# Autodesk Inventor assembly: 00_Linear_rail_X
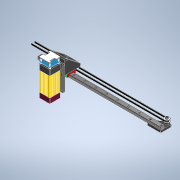
[picture p0: Inventor's stored thumbnail of the model, 180x180]
Saved by Autodesk Inventor 2022.2 (Build 262287010, 287A)
## iProperties
Created: 2022-05-03
Part Number: 00_Linear_rail_X
Document SubType Name: Assembly
Designer: MXBD
Author: MXBD
## Documents named in this file (13)
- D:\Laser_Engraver\CAD\Assembly\00_Linear_rail_X.iam
- D:\Laser_Engraver\CAD\Parts\02_mgn15h_Rail_450mm.ipt
- D:\Laser_Engraver\CAD\Parts\01_mgn15h_Bearing_Block.ipt
- D:\Laser_Engraver\CAD\Assembly\01_Laser_Assy.iam
- D:\Laser_Engraver\CAD\Parts\21_X_Pulley_holder.ipt
- D:\Laser_Engraver\CAD\Parts\23_Spacers_7.7mm.ipt
- D:\Laser_Engraver\CAD\Parts\10_GT2_Idler_Pulley_20_Teeth.ipt
- C:\Users\49152\Documents\Inventor\Content Center Files\R2022\de-DE\ISO 4762(2)\ISO 4762 - M5 x 30ISO.ipt
- C:\Users\49152\Documents\Inventor\Content Center Files\R2022\de-DE\ISO 4762(2)\ISO 4762 - M3 x 12ISO.ipt
- C:\Users\49152\Documents\Inventor\Content Center Files\R2022\de-DE\DIN 555\DIN 555-5 - M5.ipt
- C:\Users\49152\Documents\Inventor\Content Center Files\R2022\de-DE\ISO 4762(2)\ISO 4762 - M5 x 20ISO.ipt
- C:\Users\49152\Documents\Inventor\Content Center Files\R2022\de-DE\ISO 4762(2)\ISO 4762 - M3 x 8ISO.ipt
- D:\Laser_Engraver\CAD\Parts\20_Belt_490mm.ipt
## Components (18 placed, 12 different names)
1. 02_mgn15h_Rail_450mm:1 — Passend:1, Passend:2, Passend:6, Passend:7, Passend:8, Passend:15, Passend:16, Passend:17, Passend:18, Winkel:1, Passend:33, Fluchtend:1
2. 01_mgn15h_Bearing_Block:1 — Passend:1, Passend:2, Passend:3, Passend:4, Passend:5
3. 01_Laser_Assy:1 [sub-assembly] — Passend:3, Passend:4, Passend:5, Passend:21, Passend:22, Passend:23, Passend:24, Passend:25, Passend:26, Passend:27, Passend:28, Passend:29, Passend:30, Passend:31, Passend:32
4. 21_X_Pulley_holder:1 — Passend:6, Passend:7, Passend:8, Passend:9, Passend:10, Passend:20
5. 23_Spacers_7.7mm:1 — Passend:9, Passend:10, Passend:11, Passend:12
6. 10_GT2_Idler_Pulley_20_Teeth:1 — Passend:11, Passend:12, Passend:13, Passend:14, Passend:34
7. ISO 4762 M5 x 30:1 — Passend:13, Passend:14, Passend:19
8. ISO 4762 M3 x 12:1 — Passend:15, Passend:18
9. ISO 4762 M3 x 12:2 — Passend:16, Passend:17
10. DIN 555 - ersetzt durch DIN EN 24034 M5:1 — Passend:19, Passend:20
11. ISO 4762 M5 x 20:1 — Passend:21, Passend:23
12. ISO 4762 M5 x 20:2 — Passend:22, Passend:24
13. ISO 4762 M3 x 8:1 — Passend:25, Passend:31
14. ISO 4762 M3 x 8:2 — Passend:26, Passend:30
15. ISO 4762 M3 x 8:3 — Passend:27, Passend:32
16. ISO 4762 M3 x 8:4 — Passend:28, Passend:29
17. 20_Belt_490mm:2 — Passend:35, Fluchtend:2, Fluchtend:3
18. 20_Belt_490mm:3 — Winkel:1, Passend:33, Passend:34, Fluchtend:1, Passend:35, Fluchtend:2, Fluchtend:3
## Relationships (39: Mate 35, Flush 3, Angle 1)
- Passend:1 [Mate]: 02_mgn15h_Rail_450mm:1 ↔ 01_mgn15h_Bearing_Block:1
- Passend:2 [Mate]: 02_mgn15h_Rail_450mm:1 ↔ 01_mgn15h_Bearing_Block:1
- Passend:3 [Mate]: 01_mgn15h_Bearing_Block:1 ↔ 01_Laser_Assy:1
- Passend:4 [Mate]: 01_mgn15h_Bearing_Block:1 ↔ 01_Laser_Assy:1
- Passend:5 [Mate]: 01_mgn15h_Bearing_Block:1 ↔ 01_Laser_Assy:1
- Passend:6 [Mate]: 02_mgn15h_Rail_450mm:1 ↔ 21_X_Pulley_holder:1
- Passend:7 [Mate]: 02_mgn15h_Rail_450mm:1 ↔ 21_X_Pulley_holder:1
- Passend:8 [Mate]: 02_mgn15h_Rail_450mm:1 ↔ 21_X_Pulley_holder:1
- Passend:9 [Mate]: 21_X_Pulley_holder:1 ↔ 23_Spacers_7.7mm:1
- Passend:10 [Mate]: 21_X_Pulley_holder:1 ↔ 23_Spacers_7.7mm:1
- Passend:11 [Mate]: 23_Spacers_7.7mm:1 ↔ 10_GT2_Idler_Pulley_20_Teeth:1
- Passend:12 [Mate]: 23_Spacers_7.7mm:1 ↔ 10_GT2_Idler_Pulley_20_Teeth:1
- Passend:13 [Mate]: 10_GT2_Idler_Pulley_20_Teeth:1 ↔ ISO 4762 M5 x 30:1
- Passend:14 [Mate]: 10_GT2_Idler_Pulley_20_Teeth:1 ↔ ISO 4762 M5 x 30:1
- Passend:15 [Mate]: 02_mgn15h_Rail_450mm:1 ↔ ISO 4762 M3 x 12:1
- Passend:16 [Mate]: 02_mgn15h_Rail_450mm:1 ↔ ISO 4762 M3 x 12:2
- Passend:17 [Mate]: 02_mgn15h_Rail_450mm:1 ↔ ISO 4762 M3 x 12:2
- Passend:18 [Mate]: 02_mgn15h_Rail_450mm:1 ↔ ISO 4762 M3 x 12:1
- Passend:19 [Mate]: ISO 4762 M5 x 30:1 ↔ DIN 555 - ersetzt durch DIN EN 24034 M5:1
- Passend:20 [Mate]: 21_X_Pulley_holder:1 ↔ DIN 555 - ersetzt durch DIN EN 24034 M5:1
- Passend:21 [Mate]: 01_Laser_Assy:1 ↔ ISO 4762 M5 x 20:1
- Passend:22 [Mate]: 01_Laser_Assy:1 ↔ ISO 4762 M5 x 20:2
- Passend:23 [Mate]: 01_Laser_Assy:1 ↔ ISO 4762 M5 x 20:1
- Passend:24 [Mate]: 01_Laser_Assy:1 ↔ ISO 4762 M5 x 20:2
- Passend:25 [Mate]: 01_Laser_Assy:1 ↔ ISO 4762 M3 x 8:1
- Passend:26 [Mate]: 01_Laser_Assy:1 ↔ ISO 4762 M3 x 8:2
- Passend:27 [Mate]: 01_Laser_Assy:1 ↔ ISO 4762 M3 x 8:3
- Passend:28 [Mate]: 01_Laser_Assy:1 ↔ ISO 4762 M3 x 8:4
- Passend:29 [Mate]: 01_Laser_Assy:1 ↔ ISO 4762 M3 x 8:4
- Passend:30 [Mate]: 01_Laser_Assy:1 ↔ ISO 4762 M3 x 8:2
- Passend:31 [Mate]: 01_Laser_Assy:1 ↔ ISO 4762 M3 x 8:1
- Passend:32 [Mate]: 01_Laser_Assy:1 ↔ ISO 4762 M3 x 8:3
- Winkel:1 [Angle] (0 deg): 02_mgn15h_Rail_450mm:1 ↔ 20_Belt_490mm:3
- Passend:33 [Mate] (10.5 mm): 02_mgn15h_Rail_450mm:1 ↔ 20_Belt_490mm:3
- Passend:34 [Mate]: 10_GT2_Idler_Pulley_20_Teeth:1 ↔ 20_Belt_490mm:3
- Fluchtend:1 [Flush] (10 mm): 02_mgn15h_Rail_450mm:1 ↔ 20_Belt_490mm:3
- Passend:35 [Mate] (11 mm): 20_Belt_490mm:2 ↔ 20_Belt_490mm:3
- Fluchtend:2 [Flush]: 20_Belt_490mm:2 ↔ 20_Belt_490mm:3
- Fluchtend:3 [Flush]: 20_Belt_490mm:2 ↔ 20_Belt_490mm:3
